# Autodesk Inventor assembly: mecanismo
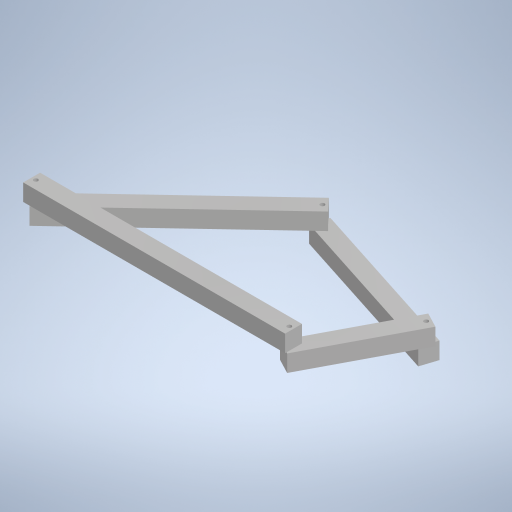
[picture p0: Inventor's stored thumbnail of the model, 512x512]
Saved by Autodesk Inventor 2023 (Build 270158000, 158)
## iProperties
Created: 2022-10-09
Part Number: mecanismo
Document SubType Name: Assembly
Designer: Administrator
Title: mecanismo v12
Author: Administrator
## Documents named in this file (5)
- C:\Users\klebe\OneDrive\Área de Trabalho\mecanismo v11\mecanismo.iam
- C:\Users\klebe\OneDrive\Área de Trabalho\mecanismo v11\Component1.ipt
- C:\Users\klebe\OneDrive\Área de Trabalho\mecanismo v11\Component2.ipt
- C:\Users\klebe\OneDrive\Área de Trabalho\mecanismo v11\Component4.ipt
- C:\Users\klebe\OneDrive\Área de Trabalho\mecanismo v11\Component5.ipt
## Components (4 placed, 4 different names)
1. Component1:1 — Rotational:1, Rotational:3
2. Component2:1 — Rotational:1, Rotational:2
3. Component4:1 — Rotational:3, Rotational:4
4. Component5:1 — Rotational:2, Rotational:4
## Relationships (4: RevoluteJoint 4)
- Rotational:1 [RevoluteJoint]: Component1:1 ↔ Component2:1
- Rotational:2 [RevoluteJoint]: Component2:1 ↔ Component5:1
- Rotational:3 [RevoluteJoint]: Component1:1 ↔ Component4:1
- Rotational:4 [RevoluteJoint]: Component4:1 ↔ Component5:1
